# Autodesk Inventor assembly: BearingDTAssembly-1111-2017
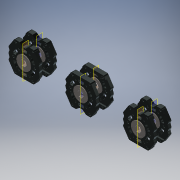
[picture p0: Inventor's stored thumbnail of the model, 180x180]
Saved by Autodesk Inventor 2017 (Build 210142000, 142)
## iProperties
Created: 2017-12-22
Part Number: BearingDTAssembly-1111-2017
Document SubType Name: Assembly
Designer: 600086
Author: 600086
## Documents named in this file (2)
- E:\2017-2018 Resources\Resources\Assembled Resources\BearingDTAssembly-1111-2017.iam
- H:\Documents\Robotics\2017-2018 PracticeChassis\Assemblies\BearingBlockAssembly-1111-2017.iam
## Components (6 placed, 1 different names)
1. BearingBlockAssembly-1111-2017:1 [sub-assembly] — Rotational:1, Mate:1
2. BearingBlockAssembly-1111-2017:2 [sub-assembly] — Rotational:1, Flush:2, Flush:5
3. BearingBlockAssembly-1111-2017:3 [sub-assembly] — Rigid:2, Flush:6, Mate:2
4. BearingBlockAssembly-1111-2017:4 [sub-assembly] — Rigid:2, Flush:4
5. BearingBlockAssembly-1111-2017:5 [sub-assembly] — Rigid:1, Flush:2, Flush:4, Flush:5
6. BearingBlockAssembly-1111-2017:6 [sub-assembly] — Rigid:1, Flush:6, Mate:1, Mate:2
## Relationships (9: Flush 4, WeldJoint 2, Mate 2, RevoluteJoint 1)
- Rotational:1 [RevoluteJoint] (25.4 mm): BearingBlockAssembly-1111-2017:1 ↔ BearingBlockAssembly-1111-2017:2
- Rigid:1 [WeldJoint] (25.4 mm): BearingBlockAssembly-1111-2017:5 ↔ BearingBlockAssembly-1111-2017:6
- Rigid:2 [WeldJoint] (25.4 mm): BearingBlockAssembly-1111-2017:3 ↔ BearingBlockAssembly-1111-2017:4
- Flush:2: BearingBlockAssembly-1111-2017:2 ↔ BearingBlockAssembly-1111-2017:5
- Flush:4: BearingBlockAssembly-1111-2017:4 ↔ BearingBlockAssembly-1111-2017:5
- Flush:5: BearingBlockAssembly-1111-2017:2 ↔ BearingBlockAssembly-1111-2017:5
- Flush:6: BearingBlockAssembly-1111-2017:3 ↔ BearingBlockAssembly-1111-2017:6
- Mate:1 (127 mm): BearingBlockAssembly-1111-2017:1 ↔ BearingBlockAssembly-1111-2017:6
- Mate:2 (-127 mm): BearingBlockAssembly-1111-2017:3 ↔ BearingBlockAssembly-1111-2017:6
